# Autodesk Inventor assembly: pelican_electronics_asm
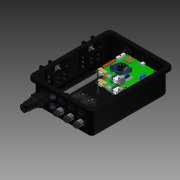
[picture p0: Inventor's stored thumbnail of the model, 180x180]
Saved by Autodesk Inventor 2016 (Build 200138000, 138)
## iProperties
Created: 2016-04-02
Part Number: pelican_electronics_asm
Document SubType Name: Assembly
Designer: hwasserb
Author: hwasserb
## Documents named in this file (23)
- C:\Users\Haden\Desktop\Cad-Model\Pelican Case\Pelican Case.iam
- C:\Users\Haden\Desktop\Cad-Model\Pelican Case\1400_BOTTOM.ipt
- C:\Users\Haden\Desktop\Cad-Model\Pelican Case\STANDOFF_4-40X1-1_2.ipt
- C:\Users\Haden\Desktop\Cad-Model\Pelican Case\RA_BARREL.ipt
- C:\Users\Haden\Desktop\Cad-Model\Pelican Case\BS2302.ipt
- C:\Users\Haden\Desktop\Cad-Model\Pelican Case\15600-06-20.ipt
- C:\Users\Haden\Desktop\Cad-Model\Pelican Case\TALON_SRX.ipt
- C:\Users\Haden\Desktop\Cad-Model\Pelican Case\RJ45-PASSTHROUGH.ipt
- C:\Users\Haden\Desktop\Cad-Model\Pelican Case\DT04-4P-L012.ipt
- C:\Users\Haden\Desktop\Cad-Model\Pelican Case\DT06-4S.ipt
- C:\Users\Haden\Desktop\Cad-Model\Pelican Case\WPUSBAX-MA1.ipt
- C:\Users\Haden\Desktop\Cad-Model\Pelican Case\SK2-050B04.ipt
- C:\Users\Haden\Desktop\Cad-Model\Pelican Case\SK6-050B04.ipt
- C:\Users\Haden\Desktop\Cad-Model\Pelican Case\1400_TOP.ipt
- C:\Users\Haden\Desktop\Cad-Model\Pelican Case\BOLT_10-32X1-1_4.ipt
- C:\Users\Haden\Desktop\Cad-Model\Pelican Case\BOLT_10-32X1.ipt
- C:\Users\Haden\Desktop\Cad-Model\Pelican Case\BOLT_8-32X1-3_8.ipt
- C:\Users\Haden\Desktop\Cad-Model\Pelican Case\BOLT_4-40X3_4.ipt
- C:\Users\Haden\Desktop\Cad-Model\Pelican Case\BOLT_8-32X3_4.ipt
- C:\Users\Haden\Desktop\Cad-Model\Pelican Case\BOLT_4-40X1_4.ipt
- C:\Users\Haden\Desktop\Cad-Model\Pelican Case\Jetson TK1\Jetson TK1.iam
- C:\Users\Haden\Desktop\Cad-Model\Pelican Case\Interfacer\Interfacer.iam
- C:\Users\Haden\Desktop\Cad-Model\Pelican Case\Netgear GS105 Enet Switch\Netgear GS105 Enet Switch.iam
## Components (69 placed, 22 different names)
1. 1400_BOTTOM:1 — Insert:1, Insert:2, Insert:3, Insert:4, Insert:5, Insert:6, Insert:7, Insert:8, Insert:9, Insert:10, Insert:11, Insert:12, Insert:13, Insert:14, Insert:15, Insert:16, Insert:17, Insert:18, Insert:19, Insert:20, Insert:21, Insert:22, Insert:23, Insert:24, Insert:25, Insert:26, Insert:27, Insert:28, Insert:29, Insert:30, Insert:31, Insert:32, Insert:33, Insert:34, Insert:35, Insert:36, Angle:2, Mate:1, Mate:2, Mate:3, Insert:49, Insert:50, Insert:51, Insert:52, Insert:53, Insert:54, Insert:55, Insert:56, Insert:57, Insert:58, Insert:59, Insert:60, Insert:61, Insert:62, Insert:63, Insert:64, Insert:65, Insert:66, Insert:67, Insert:68
2. STANDOFF_4-40X1-1_2:1 — Insert:31, Flush:4, Insert:37
3. STANDOFF_4-40X1-1_2:2 — Insert:32, Flush:3
4. STANDOFF_4-40X1-1_2:3 — Insert:29, Flush:2
5. STANDOFF_4-40X1-1_2:4 — Insert:30, Flush:1, Insert:38
6. STANDOFF_4-40X1-1_2:5 — Flush:4, Flush:5, Angle:1, Angle:2, Insert:40, Insert:44
7. STANDOFF_4-40X1-1_2:6 — Flush:3, Flush:6, Angle:1, Insert:42
8. STANDOFF_4-40X1-1_2:7 — Flush:2, Flush:6, Insert:41
9. STANDOFF_4-40X1-1_2:8 — Flush:1, Flush:5, Insert:39, Insert:43
10. RA_BARREL:1
11. RA_BARREL:2
12. BS2302:1 — Insert:15, Insert:16
13. 15600-06-20:1 — Insert:3, Insert:4
14. 15600-06-20:2 — Insert:5, Insert:6
15. TALON_SRX:1 — Insert:23, Insert:24
16. TALON_SRX:2 — Insert:19, Insert:20
17. RJ45-PASSTHROUGH:1
18. RJ45-PASSTHROUGH:2
19. RJ45-PASSTHROUGH:3
20. RJ45-PASSTHROUGH:4
21. DT04-4P-L012:1 — Insert:53, Insert:54
22. DT04-4P-L012:2 — Insert:51, Insert:52
23. DT04-4P-L012:3 — Insert:49, Insert:50
24. DT06-4S:1
25. DT06-4S:2
26. DT06-4S:3
27. WPUSBAX-MA1:1
28. WPUSBAX-MA1:2
29. SK2-050B04:1 — Insert:67, Insert:68
30. SK6-050B04:1
31. 1400_TOP:1
32. BOLT_10-32X1-1_4:1 — Insert:7
33. BOLT_10-32X1-1_4:2 — Insert:9
34. BOLT_10-32X1-1_4:3 — Insert:10
35. BOLT_10-32X1-1_4:4 — Insert:8
36. BOLT_10-32X1-1_4:5 — Insert:13
37. BOLT_10-32X1-1_4:6 — Insert:14
38. BOLT_10-32X1-1_4:7 — Insert:11
39. BOLT_10-32X1-1_4:8 — Insert:12
40. BOLT_10-32X1:1 — Insert:18
41. BOLT_10-32X1:2 — Insert:17
42. BOLT_8-32X1-3_8:1 — Insert:26
43. BOLT_8-32X1-3_8:2 — Insert:28
44. BOLT_8-32X1-3_8:3 — Insert:27
45. BOLT_8-32X1-3_8:4 — Insert:25
46. BOLT_4-40X3_4:1 — Insert:36
47. BOLT_4-40X3_4:2 — Insert:33
48. BOLT_4-40X3_4:3 — Insert:34
49. BOLT_4-40X3_4:4 — Insert:35
50. BOLT_8-32X3_4:1 — Insert:56
51. BOLT_8-32X3_4:2 — Insert:66
52. BOLT_8-32X3_4:3 — Insert:65
53. BOLT_8-32X3_4:4 — Insert:64
54. BOLT_8-32X3_4:5 — Insert:63
55. BOLT_8-32X3_4:6 — Insert:62
56. BOLT_8-32X3_4:7 — Insert:61
57. BOLT_8-32X3_4:8 — Insert:60
58. BOLT_8-32X3_4:9 — Insert:59
59. BOLT_8-32X3_4:10 — Insert:55
60. BOLT_8-32X3_4:11 — Insert:58
61. BOLT_8-32X3_4:12 — Insert:57
62. BOLT_4-40X1_4:1 — Insert:46
63. BOLT_4-40X1_4:2 — Insert:45
64. BOLT_4-40X1_4:3 — Insert:47
65. BOLT_4-40X1_4:4 — Insert:48
66. Jetson TK1:1 [sub-assembly] — Insert:43, Insert:44, Insert:45, Insert:46, Insert:47, Insert:48
67. Jetson TK1:2 [sub-assembly] — Insert:37, Insert:38, Insert:39, Insert:40, Insert:41, Insert:42
68. Interfacer:1 [sub-assembly] — Insert:1, Insert:2, Insert:21, Insert:22
69. Netgear GS105 Enet Switch:1 [sub-assembly] — Mate:1, Mate:2, Mate:3
## Relationships (79: Insert 68, Flush 6, Mate 3, Angle 2)
- Insert:1: 1400_BOTTOM:1 ↔ Interfacer:1
- Insert:2: 1400_BOTTOM:1 ↔ Interfacer:1
- Insert:3: 1400_BOTTOM:1 ↔ 15600-06-20:1
- Insert:4: 1400_BOTTOM:1 ↔ 15600-06-20:1
- Insert:5: 1400_BOTTOM:1 ↔ 15600-06-20:2
- Insert:6: 1400_BOTTOM:1 ↔ 15600-06-20:2
- Insert:7: 1400_BOTTOM:1 ↔ BOLT_10-32X1-1_4:1
- Insert:8: 1400_BOTTOM:1 ↔ BOLT_10-32X1-1_4:4
- Insert:9: 1400_BOTTOM:1 ↔ BOLT_10-32X1-1_4:2
- Insert:10: 1400_BOTTOM:1 ↔ BOLT_10-32X1-1_4:3
- Insert:11: 1400_BOTTOM:1 ↔ BOLT_10-32X1-1_4:7
- Insert:12: 1400_BOTTOM:1 ↔ BOLT_10-32X1-1_4:8
- Insert:13: 1400_BOTTOM:1 ↔ BOLT_10-32X1-1_4:5
- Insert:14: 1400_BOTTOM:1 ↔ BOLT_10-32X1-1_4:6
- Insert:15: 1400_BOTTOM:1 ↔ BS2302:1
- Insert:16: 1400_BOTTOM:1 ↔ BS2302:1
- Insert:17: 1400_BOTTOM:1 ↔ BOLT_10-32X1:2
- Insert:18: 1400_BOTTOM:1 ↔ BOLT_10-32X1:1
- Insert:19: 1400_BOTTOM:1 ↔ TALON_SRX:2
- Insert:20: 1400_BOTTOM:1 ↔ TALON_SRX:2
- Insert:21: 1400_BOTTOM:1 ↔ Interfacer:1
- Insert:22: 1400_BOTTOM:1 ↔ Interfacer:1
- Insert:23: 1400_BOTTOM:1 ↔ TALON_SRX:1
- Insert:24: 1400_BOTTOM:1 ↔ TALON_SRX:1
- Insert:25: 1400_BOTTOM:1 ↔ BOLT_8-32X1-3_8:4
- Insert:26: 1400_BOTTOM:1 ↔ BOLT_8-32X1-3_8:1
- Insert:27: 1400_BOTTOM:1 ↔ BOLT_8-32X1-3_8:3
- Insert:28: 1400_BOTTOM:1 ↔ BOLT_8-32X1-3_8:2
- Insert:29: 1400_BOTTOM:1 ↔ STANDOFF_4-40X1-1_2:3
- Insert:30: 1400_BOTTOM:1 ↔ STANDOFF_4-40X1-1_2:4
- Insert:31: 1400_BOTTOM:1 ↔ STANDOFF_4-40X1-1_2:1
- Insert:32: 1400_BOTTOM:1 ↔ STANDOFF_4-40X1-1_2:2
- Insert:33: 1400_BOTTOM:1 ↔ BOLT_4-40X3_4:2
- Insert:34: 1400_BOTTOM:1 ↔ BOLT_4-40X3_4:3
- Insert:35: 1400_BOTTOM:1 ↔ BOLT_4-40X3_4:4
- Insert:36: 1400_BOTTOM:1 ↔ BOLT_4-40X3_4:1
- Flush:1: STANDOFF_4-40X1-1_2:4 ↔ STANDOFF_4-40X1-1_2:8
- Flush:2: STANDOFF_4-40X1-1_2:3 ↔ STANDOFF_4-40X1-1_2:7
- Flush:3: STANDOFF_4-40X1-1_2:2 ↔ STANDOFF_4-40X1-1_2:6
- Flush:4: STANDOFF_4-40X1-1_2:1 ↔ STANDOFF_4-40X1-1_2:5
- Flush:5: STANDOFF_4-40X1-1_2:5 ↔ STANDOFF_4-40X1-1_2:8
- Flush:6: STANDOFF_4-40X1-1_2:6 ↔ STANDOFF_4-40X1-1_2:7
- Angle:1 (0 deg): STANDOFF_4-40X1-1_2:5 ↔ STANDOFF_4-40X1-1_2:6
- Angle:2 (0 deg): 1400_BOTTOM:1 ↔ STANDOFF_4-40X1-1_2:5
- Mate:1: 1400_BOTTOM:1 ↔ Netgear GS105 Enet Switch:1
- Mate:2: 1400_BOTTOM:1 ↔ Netgear GS105 Enet Switch:1
- Insert:37: STANDOFF_4-40X1-1_2:1 ↔ Jetson TK1:2
- Insert:38: STANDOFF_4-40X1-1_2:4 ↔ Jetson TK1:2
- Mate:3: 1400_BOTTOM:1 ↔ Netgear GS105 Enet Switch:1
- Insert:39: STANDOFF_4-40X1-1_2:8 ↔ Jetson TK1:2
- Insert:40: STANDOFF_4-40X1-1_2:5 ↔ Jetson TK1:2
- Insert:41: STANDOFF_4-40X1-1_2:7 ↔ Jetson TK1:2
- Insert:42: STANDOFF_4-40X1-1_2:6 ↔ Jetson TK1:2
- Insert:43: STANDOFF_4-40X1-1_2:8 ↔ Jetson TK1:1
- Insert:44: STANDOFF_4-40X1-1_2:5 ↔ Jetson TK1:1
- Insert:45: BOLT_4-40X1_4:2 ↔ Jetson TK1:1
- Insert:46: BOLT_4-40X1_4:1 ↔ Jetson TK1:1
- Insert:47: BOLT_4-40X1_4:3 ↔ Jetson TK1:1
- Insert:48: BOLT_4-40X1_4:4 ↔ Jetson TK1:1
- Insert:49: 1400_BOTTOM:1 ↔ DT04-4P-L012:3
- Insert:50: 1400_BOTTOM:1 ↔ DT04-4P-L012:3
- Insert:51: 1400_BOTTOM:1 ↔ DT04-4P-L012:2
- Insert:52: 1400_BOTTOM:1 ↔ DT04-4P-L012:2
- Insert:53: 1400_BOTTOM:1 ↔ DT04-4P-L012:1
- Insert:54: 1400_BOTTOM:1 ↔ DT04-4P-L012:1
- Insert:55: 1400_BOTTOM:1 ↔ BOLT_8-32X3_4:10
- Insert:56: 1400_BOTTOM:1 ↔ BOLT_8-32X3_4:1
- Insert:57: 1400_BOTTOM:1 ↔ BOLT_8-32X3_4:12
- Insert:58: 1400_BOTTOM:1 ↔ BOLT_8-32X3_4:11
- Insert:59: 1400_BOTTOM:1 ↔ BOLT_8-32X3_4:9
- Insert:60: 1400_BOTTOM:1 ↔ BOLT_8-32X3_4:8
- Insert:61: 1400_BOTTOM:1 ↔ BOLT_8-32X3_4:7
- Insert:62: 1400_BOTTOM:1 ↔ BOLT_8-32X3_4:6
- Insert:63: 1400_BOTTOM:1 ↔ BOLT_8-32X3_4:5
- Insert:64: 1400_BOTTOM:1 ↔ BOLT_8-32X3_4:4
- Insert:65: 1400_BOTTOM:1 ↔ BOLT_8-32X3_4:3
- Insert:66: 1400_BOTTOM:1 ↔ BOLT_8-32X3_4:2
- Insert:67: 1400_BOTTOM:1 ↔ SK2-050B04:1
- Insert:68: 1400_BOTTOM:1 ↔ SK2-050B04:1
